# Autodesk Inventor assembly: centric_shaft_controller_smaller
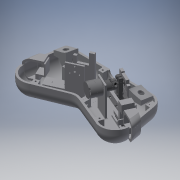
[picture p0: Inventor's stored thumbnail of the model, 180x180]
Saved by Autodesk Inventor 2016 (Build 200138000, 138)
## iProperties
Created: 2018-03-13
Part Number: centric_shaft_controller_smaller
Document SubType Name: Assembly
Designer: oechslin
Author: oechslin
## Documents named in this file (10)
- C:\Users\oechslin\Documents\Inventor_workspace\20180312_centric_shaft_geometric_controller_design\centric_shaft_controller_smaller.iam
- C:\Users\oechslin\Documents\Inventor_workspace\20180312_centric_shaft_geometric_controller_design\L_js_mount.ipt
- C:\Users\oechslin\Documents\Inventor_workspace\20180312_centric_shaft_geometric_controller_design\R_js_mount.ipt
- C:\Users\oechslin\Documents\Inventor_workspace\20180312_centric_shaft_geometric_controller_design\L_palm_pad.ipt
- C:\Users\oechslin\Documents\Inventor_workspace\20180312_centric_shaft_geometric_controller_design\R_palm_pad.ipt
- C:\Users\oechslin\Documents\Inventor_workspace\20180312_centric_shaft_geometric_controller_design\R_cover.ipt
- C:\Users\oechslin\Documents\Inventor_workspace\20180312_centric_shaft_geometric_controller_design\L_cover.ipt
- C:\Users\oechslin\Documents\Inventor_workspace\20180312_centric_shaft_geometric_controller_design\R_base.ipt
- C:\Users\oechslin\Documents\Inventor_workspace\20180312_centric_shaft_geometric_controller_design\L_base.ipt
- C:\Users\oechslin\Documents\Inventor_workspace\20180312_centric_shaft_geometric_controller_design\assembly_motor_right.iam
## Components (9 placed, 9 different names)
1. L_js_mount:1
2. R_js_mount:1
3. L_palm_pad:1
4. R_palm_pad:1 — Mate:5
5. R_cover:1
6. L_cover:1
7. R_base:1 — Mate:1, Mate:2, Mate:3, Mate:4, Flush:1
8. L_base:1
9. assembly_motor_right:1 [sub-assembly] — Mate:1, Mate:2, Mate:3, Mate:4, Flush:1, Mate:5
## Relationships (6: Mate 5, Flush 1)
- Mate:1: R_base:1 ↔ assembly_motor_right:1
- Mate:2: R_base:1 ↔ assembly_motor_right:1
- Mate:3: R_base:1 ↔ assembly_motor_right:1
- Mate:4: R_base:1 ↔ assembly_motor_right:1
- Flush:1 (6 mm): R_base:1 ↔ assembly_motor_right:1
- Mate:5 (5 mm): R_palm_pad:1 ↔ assembly_motor_right:1
